# Autodesk Inventor assembly: Motor+Pantilt
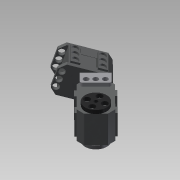
[picture p0: Inventor's stored thumbnail of the model, 180x180]
Saved by Autodesk Inventor 2014 (Build 180170000, 170)
## iProperties
Created: 2014-03-07
Part Number: Motor+Pantilt
Document SubType Name: Assembly
Designer: Grégoire
Author: Grégoire
## Documents named in this file (5)
- C:\Users\Grégoire\Desktop\XL320\src\Motor+Pantilt.iam
- C:\Users\Grégoire\Desktop\XL320\src\Motor.ipt
- C:\Users\Grégoire\Desktop\XL320\src\Arm.ipt
- C:\Users\Grégoire\Desktop\XL320\src\CounterArm.ipt
- C:\Users\Grégoire\Desktop\XL320\src\Pantilt.ipt
## Components (7 placed, 4 different names)
1. Motor:1 — Placage:1, Placage:2, Placage:3, Placage:4
2. Arm:1 — Placage:3, Placage:4, Placage:9, Placage:10, Placage:11
3. CounterArm:1 — Placage:1, Placage:2
4. Motor:2 — Placage:12, Placage:14, Placage:15
5. Arm:2
6. CounterArm:2
7. Pantilt:1 — Placage:9, Placage:10, Placage:11, Placage:12, Placage:14, Placage:15
## Relationships (14: Mate 14)
- Placage:1 [Mate]: Motor:1 ↔ CounterArm:1
- Placage:2 [Mate]: Motor:1 ↔ CounterArm:1
- Placage:3 [Mate]: Motor:1 ↔ Arm:1
- Placage:4 [Mate]: Motor:1 ↔ Arm:1
- [Mate]: Motor:2 ↔ CounterArm:2
- [Mate]: Motor:2 ↔ CounterArm:2
- [Mate]: Motor:2 ↔ Arm:2
- [Mate]: Motor:2 ↔ Arm:2
- Placage:9 [Mate]: Arm:1 ↔ Pantilt:1
- Placage:10 [Mate]: Arm:1 ↔ Pantilt:1
- Placage:11 [Mate]: Arm:1 ↔ Pantilt:1
- Placage:12 [Mate]: Motor:2 ↔ Pantilt:1
- Placage:14 [Mate]: Motor:2 ↔ Pantilt:1
- Placage:15 [Mate]: Motor:2 ↔ Pantilt:1
## Named parameters: d20_d0 = 0 mm, d21_d1 = 0 mm, d22_d2 = 0 mm, d23_d3 = 0 mm
